# Autodesk Inventor assembly: main_board
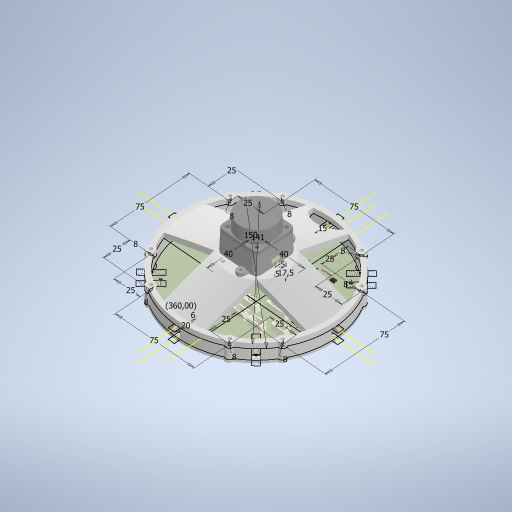
[picture p0: Inventor's stored thumbnail of the model, 512x512]
Saved by Autodesk Inventor 2024.3 (Build 283343000, 343)
## iProperties
Created: 2026-05-02
Part Number: main_board
Document SubType Name: Assembly
Designer: owozn
Author: owozn
## Documents named in this file (5)
- C:\Users\owozn\Documents\Nauka\Studia\mgr\Semestr_3\Magisterka\uMule\mechanics\subsets\attachments\main_board\main_board.iam
- C:\Users\owozn\Documents\Nauka\Studia\mgr\Semestr_3\Magisterka\uMule\mechanics\subsets\attachments\main_board\board_holder.ipt
- C:\Users\owozn\Documents\Nauka\Studia\mgr\Semestr_3\Magisterka\uMule\mechanics\subsets\attachments\main_board\uMule_board\uMule_board.iam
- C:\Users\owozn\Documents\Nauka\Studia\mgr\Semestr_3\Magisterka\uMule\mechanics\subsets\attachments\lidar\lidar_holder.ipt
- C:\Users\owozn\Documents\Nauka\Studia\mgr\Semestr_3\Magisterka\uMule\mechanics\subsets\attachments\lidar\LD19_v2\STL-19P_LiDaRLD19_v2.iam
## Components (4 placed, 4 different names)
1. board_holder:1 — Mate:1, Mate:2, Mate:3, Mate:4, Mate:5
2. uMule_board:1 [sub-assembly] — Mate:1, Mate:2
3. lidar_holder:1 — Mate:3, Mate:4, Mate:5, Mate:6, Mate:7, Mate:8
4. STL-19P_LiDaRLD19_v2:1 [sub-assembly] — Mate:6, Mate:7, Mate:8
## Relationships (8: Mate 8)
- Mate:1: board_holder:1 ↔ uMule_board:1
- Mate:2: board_holder:1 ↔ uMule_board:1
- Mate:3: board_holder:1 ↔ lidar_holder:1
- Mate:4: board_holder:1 ↔ lidar_holder:1
- Mate:5: board_holder:1 ↔ lidar_holder:1
- Mate:6: lidar_holder:1 ↔ STL-19P_LiDaRLD19_v2:1
- Mate:7: lidar_holder:1 ↔ STL-19P_LiDaRLD19_v2:1
- Mate:8: lidar_holder:1 ↔ STL-19P_LiDaRLD19_v2:1
